# Autodesk Inventor assembly: Analisis_brazo
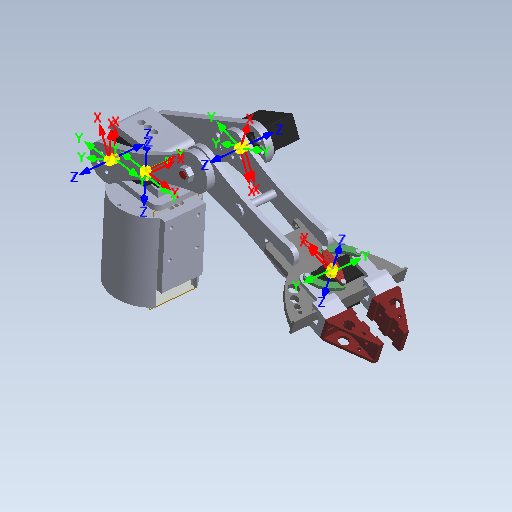
[picture p0: Inventor's stored thumbnail of the model, 512x512]
Saved by Autodesk Inventor 2020 (Build 240168000, 168)
## iProperties
Created: 2018-10-20
Part Number: Analisis_brazo
Material: Типовые
Document SubType Name: Assembly
Designer: ISULAB
Sending System: SolidWorks 2018
Last Author: E_A
Last Saved: 2018-12-07
Author: ISULAB
## Documents named in this file (17)
- D:\Документы\Рабочий стол\Артур\Модели роботов\Мобильный манипулятор\Модель\Детали\Манипулятор\Analisis_brazo.iam
- D:\Документы\Рабочий стол\Артур\Модели роботов\Мобильный манипулятор\Модель\Компоненты\3.MotorMG996R.ipt
- D:\Документы\Рабочий стол\Артур\Модели роботов\Мобильный манипулятор\Модель\Детали\Манипулятор\brazo_1.ipt
- D:\Документы\Рабочий стол\Артур\Модели роботов\Мобильный манипулятор\Модель\Детали\Манипулятор\brazo_2.ipt
- D:\Документы\Рабочий стол\Артур\Модели роботов\Мобильный манипулятор\Модель\Детали\Манипулятор\Ensamblaje1^Analisis_brazo.iam
- D:\Документы\Рабочий стол\Артур\Модели роботов\Мобильный манипулятор\Модель\Детали\Манипулятор\Ensamblaje1.iam
- D:\Документы\Рабочий стол\Артур\Модели роботов\Мобильный манипулятор\Модель\Детали\Манипулятор\BrazoSuperior_1.ipt
- D:\Документы\Рабочий стол\Артур\Модели роботов\Мобильный манипулятор\Модель\Детали\Манипулятор\BrazoSuperior_2.ipt
- D:\Документы\Рабочий стол\Артур\Модели роботов\Мобильный манипулятор\Модель\Детали\Манипулятор\cilindro_superior.ipt
- D:\Документы\Рабочий стол\Артур\Модели роботов\Мобильный манипулятор\Модель\Детали\Манипулятор\base2.ipt
- D:\Документы\Рабочий стол\Артур\Модели роботов\Мобильный манипулятор\Модель\Детали\Манипулятор\cilindro_1.ipt
- D:\Документы\Рабочий стол\Артур\Модели роботов\Мобильный манипулятор\Модель\Детали\Манипулятор\Tuerca1.ipt
- D:\Документы\Рабочий стол\Артур\Модели роботов\Мобильный манипулятор\Модель\Детали\Манипулятор\cilindro_3.ipt
- D:\Документы\Рабочий стол\Артур\Модели роботов\Мобильный манипулятор\Модель\Детали\Манипулятор\Tuerca2.ipt
- D:\Документы\Рабочий стол\Артур\Модели роботов\Мобильный манипулятор\Модель\Детали\Манипулятор\dissta.ipt
- D:\Документы\Рабочий стол\Артур\Модели роботов\Мобильный манипулятор\Модель\Детали\Манипулятор\1.BASE_2.ipt
- D:\Документы\Рабочий стол\Артур\Модели роботов\Мобильный манипулятор\Модель\Детали\Манипулятор\Servo krepej.ipt
## Components (20 placed, 16 different names)
1. 3.MotorMG996R:1 — Жесткий:3, С поворотом:9
2. brazo_1:1 — Цилиндрический:3, С поворотом:8, Жесткий:16
3. brazo_2:1 — С поворотом:2, Жесткий:5, Жесткий:6, Цилиндрический:3
4. Ensamblaje1^Analisis_brazo:1 [sub-assembly]
5. Ensamblaje1:1 [sub-assembly] — Жесткий:15
6. 3.MotorMG996R:3 — С поворотом:10, Жесткий:20
7. 3.MotorMG996R:5 — Жесткий:6, С поворотом:11
8. BrazoSuperior_1:1 — Заподлицо:1, Заподлицо:2, Жесткий:15, Жесткий:19
9. BrazoSuperior_2:1 — Жесткий:10, С поворотом:6, С поворотом:7, С поворотом:8, Заподлицо:1, Заподлицо:2
10. cilindro_superior:1 — Жесткий:10
11. base2:1 — Жесткий:3, Жесткий:4, С поворотом:2, Жесткий:17
12. cilindro_1:1 — Жесткий:4
13. Tuerca1:2 — Жесткий:5
14. cilindro_3:1 — С поворотом:7, Жесткий:14
15. Tuerca2:1 — Жесткий:14
16. dissta:1 — С поворотом:6
17. 1.BASE_2:1 — Жесткий:20
18. Servo krepej:1 — С поворотом:9, Жесткий:16
19. Servo krepej:2 — Жесткий:17, С поворотом:10
20. Servo krepej:3 — С поворотом:11, Жесткий:19
## Relationships (21: WeldJoint 11, RevoluteJoint 7, Flush 2, CylindricalJoint 1)
- Жесткий:3 [WeldJoint]: 3.MotorMG996R:1 ↔ base2:1
- Жесткий:4 [WeldJoint]: base2:1 ↔ cilindro_1:1
- С поворотом:2 [RevoluteJoint] (1.5 mm): brazo_2:1 ↔ base2:1
- Жесткий:5 [WeldJoint]: brazo_2:1 ↔ Tuerca1:2
- Жесткий:6 [WeldJoint]: brazo_2:1 ↔ 3.MotorMG996R:5
- Жесткий:10 [WeldJoint]: BrazoSuperior_2:1 ↔ cilindro_superior:1
- С поворотом:6 [RevoluteJoint]: BrazoSuperior_2:1 ↔ dissta:1
- С поворотом:7 [RevoluteJoint] (1.5 mm): BrazoSuperior_2:1 ↔ cilindro_3:1
- Цилиндрический:3 [CylindricalJoint]: brazo_1:1 ↔ brazo_2:1
- С поворотом:8 [RevoluteJoint] (3.5 mm): brazo_1:1 ↔ BrazoSuperior_2:1
- Заподлицо:1 [Flush]: BrazoSuperior_1:1 ↔ BrazoSuperior_2:1
- Заподлицо:2 [Flush]: BrazoSuperior_1:1 ↔ BrazoSuperior_2:1
- Жесткий:14 [WeldJoint]: cilindro_3:1 ↔ Tuerca2:1
- Жесткий:15 [WeldJoint]: Ensamblaje1:1 ↔ BrazoSuperior_1:1
- С поворотом:9 [RevoluteJoint]: 3.MotorMG996R:1 ↔ Servo krepej:1
- Жесткий:16 [WeldJoint]: brazo_1:1 ↔ Servo krepej:1
- Жесткий:17 [WeldJoint]: base2:1 ↔ Servo krepej:2
- С поворотом:10 [RevoluteJoint]: 3.MotorMG996R:3 ↔ Servo krepej:2
- С поворотом:11 [RevoluteJoint]: 3.MotorMG996R:5 ↔ Servo krepej:3
- Жесткий:19 [WeldJoint]: BrazoSuperior_1:1 ↔ Servo krepej:3
- Жесткий:20 [WeldJoint]: 3.MotorMG996R:3 ↔ 1.BASE_2:1
